# Autodesk Inventor assembly: shadeAssembly
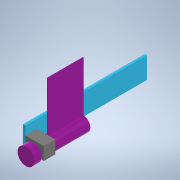
[picture p0: Inventor's stored thumbnail of the model, 180x180]
Saved by Autodesk Inventor 2021.2 (Build 252289000, 289)
## iProperties
Created: 2021-02-12
Part Number: shadeAssembly
Document SubType Name: Assembly
Designer: robst
Author: robst
## Documents named in this file (4)
- C:\git\CAD-Development\robSteele\HouseProjects\TrailerProjects\shadeAssembly.iam
- C:\git\CAD-Development\robSteele\HouseProjects\TrailerProjects\shadeHolder.ipt
- C:\git\CAD-Development\robSteele\HouseProjects\TrailerProjects\portionOfShade.ipt
- C:\git\CAD-Development\robSteele\HouseProjects\TrailerProjects\backPlate.ipt
## Components (3 placed, 3 different names)
1. shadeHolder:1 — Mate:1, Flush:1, Flush:2, Insert:1
2. portionOfShade:1 — Insert:1
3. backPlate:1 — Mate:1, Flush:1, Flush:2
## Relationships (4: Flush 2, Mate 1, Insert 1)
- Mate:1: shadeHolder:1 ↔ backPlate:1
- Flush:1: shadeHolder:1 ↔ backPlate:1
- Flush:2: shadeHolder:1 ↔ backPlate:1
- Insert:1 (1.27 mm): shadeHolder:1 ↔ portionOfShade:1
